# Autodesk Inventor assembly: Assembly2
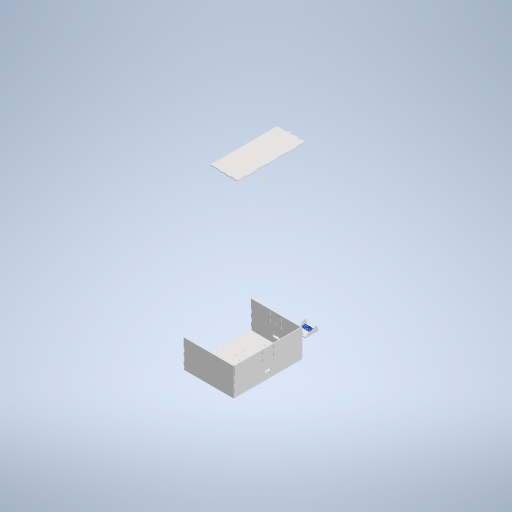
[picture p0: Inventor's stored thumbnail of the model, 512x512]
Saved by Autodesk Inventor 2023 (Build 270158000, 158)
## iProperties
Created: 2022-11-21
Part Number: Assembly2
Document SubType Name: Assembly
Designer: ADMIN
Author: ADMIN
## Documents named in this file (9)
- C:\Users\ADMIN\OneDrive\Máy tính\bản vẽ của Trung\Assembly2.iam
- C:\Users\ADMIN\OneDrive\Máy tính\bản vẽ của Trung\do_sensor_1_3mm.ipt
- C:\Users\ADMIN\OneDrive\Máy tính\bản vẽ của Trung\do_sensor_2.ipt
- C:\Users\ADMIN\OneDrive\Máy tính\bản vẽ của Trung\mieng_ben_3mm.ipt
- C:\Users\ADMIN\OneDrive\Máy tính\bản vẽ của Trung\mieng_ben_gan_sensor_3mm.ipt
- C:\Users\ADMIN\OneDrive\Máy tính\bản vẽ của Trung\mieng_mat_3mm.ipt
- C:\Users\ADMIN\OneDrive\Máy tính\bản vẽ của Trung\mieng_mat_5mm.ipt
- C:\Users\ADMIN\OneDrive\Máy tính\bản vẽ của Trung\totalPart.ipt
- C:\Users\ADMIN\OneDrive\Máy tính\bản vẽ của Trung\HC-SR04 Ultrasonic Sensor\HCSR04 Ultrasonic Sensor.ipt
## Components (9 placed, 8 different names)
1. do_sensor_1_3mm:1 — Mate:10, Mate:11, Mate:12, Mate:13, Mate:14, Mate:15, Mate:16
2. do_sensor_2:1 — Mate:13, Mate:14, Mate:15
3. mieng_ben_3mm:1
4. mieng_ben_gan_sensor_3mm:1 — Mate:7, Mate:8, Mate:9
5. mieng_mat_3mm:1 — Mate:4, Mate:5, Mate:6
6. mieng_mat_5mm:1 — Mate:1, Mate:2, Mate:3
7. totalPart:1 — Mate:1, Mate:2, Mate:3, Mate:4, Mate:5, Mate:6, Mate:7, Mate:8, Mate:9
8. do_sensor_2:2 — Mate:10, Mate:11, Mate:12
9. HCSR04 Ultrasonic Sensor:1 — Mate:16
## Relationships (16: Mate 16)
- Mate:1: mieng_mat_5mm:1 ↔ totalPart:1
- Mate:2: mieng_mat_5mm:1 ↔ totalPart:1
- Mate:3: mieng_mat_5mm:1 ↔ totalPart:1
- Mate:4: mieng_mat_3mm:1 ↔ totalPart:1
- Mate:5: mieng_mat_3mm:1 ↔ totalPart:1
- Mate:6: mieng_mat_3mm:1 ↔ totalPart:1
- Mate:7: mieng_ben_gan_sensor_3mm:1 ↔ totalPart:1
- Mate:8: mieng_ben_gan_sensor_3mm:1 ↔ totalPart:1
- Mate:9: mieng_ben_gan_sensor_3mm:1 ↔ totalPart:1
- Mate:10: do_sensor_1_3mm:1 ↔ do_sensor_2:2
- Mate:11: do_sensor_1_3mm:1 ↔ do_sensor_2:2
- Mate:12: do_sensor_1_3mm:1 ↔ do_sensor_2:2
- Mate:13: do_sensor_1_3mm:1 ↔ do_sensor_2:1
- Mate:14: do_sensor_1_3mm:1 ↔ do_sensor_2:1
- Mate:15: do_sensor_1_3mm:1 ↔ do_sensor_2:1
- Mate:16: do_sensor_1_3mm:1 ↔ HCSR04 Ultrasonic Sensor:1
